# Autodesk Inventor assembly: Shoulder
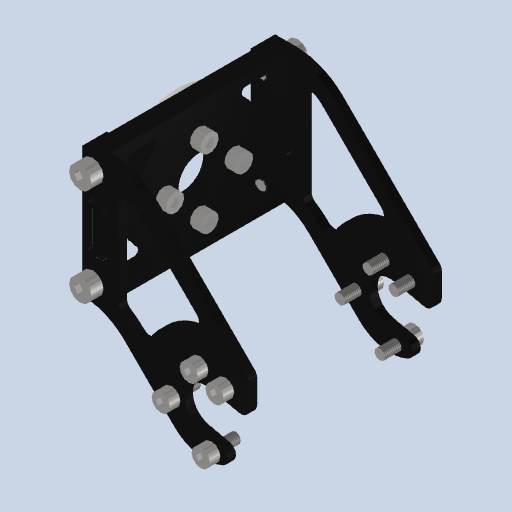
[picture p0: Inventor's stored thumbnail of the model, 512x512]
Saved by Autodesk Inventor 2022 (Build 260153000, 153)
## iProperties
Created: 2022-01-10
Part Number: Shoulder
Document SubType Name: Assembly
Designer: Masato Kubotera
Author: Masato Kubotera
## Documents named in this file (7)
- C:\Users\MasatoKubotera\Desktop\SUSTAINA-OP\UpperBody\Arm\Shoulder.iam
- C:\Users\MasatoKubotera\Desktop\SUSTAINA-OP\ReadyMade\Washer\TT-2532-10.ipt
- C:\Users\MasatoKubotera\Desktop\SUSTAINA-OP\UpperBody\Arm\Shoulder_horn_frame.ipt
- C:\Users\MasatoKubotera\Desktop\SUSTAINA-OP\UpperBody\Arm\Shoulder_side_frame.ipt
- C:\Users\MasatoKubotera\Desktop\SUSTAINA-OP\ReadyMade\Screw\UC-2606.ipt
- C:\Users\MasatoKubotera\Desktop\SUSTAINA-OP\ReadyMade\Screw\UC-2608.ipt
- C:\Users\MasatoKubotera\Desktop\SUSTAINA-OP\ReadyMade\Screw\UC-0306.ipt
## Components (20 placed, 6 different names)
1. Shoulder_horn_frame:1 — メイト:1, メイト:2, メイト:3, 挿入:1, 挿入:2, 挿入:3, 挿入:4, 挿入:5, 挿入:14, 挿入:15, 挿入:16, 挿入:17
2. Shoulder_side_frame:1 — 挿入:2, 挿入:3, 挿入:6, 挿入:7, 挿入:8, 挿入:9, 挿入:18, 挿入:19
3. Shoulder_side_frame:2 — 挿入:4, 挿入:5, 挿入:10, 挿入:11, 挿入:12, 挿入:13, 挿入:20, 挿入:21
4. TT-2532-10:1 — 挿入:1
5. UC-2606:1 — 挿入:6
6. UC-2606:2 — 挿入:7
7. UC-2606:3 — 挿入:8
8. UC-2606:4 — 挿入:9
9. UC-2606:5 — 挿入:10
10. UC-2606:6 — 挿入:11
11. UC-2606:7 — 挿入:12
12. UC-2606:8 — 挿入:13
13. UC-2608:1 — 挿入:14
14. UC-2608:2 — 挿入:15
15. UC-2608:3 — 挿入:16
16. UC-2608:4 — 挿入:17
17. UC-0306:1 — 挿入:18
18. UC-0306:2 — 挿入:19
19. UC-0306:3 — 挿入:20
20. UC-0306:4 — 挿入:21
## Relationships (24: Insert 21, Mate 3)
- メイト:1 [Mate]: Shoulder_horn_frame:1
- メイト:2 [Mate]: Shoulder_horn_frame:1
- メイト:3 [Mate]: Shoulder_horn_frame:1
- 挿入:1 [Insert]: Shoulder_horn_frame:1 ↔ TT-2532-10:1
- 挿入:2 [Insert]: Shoulder_horn_frame:1 ↔ Shoulder_side_frame:1
- 挿入:3 [Insert]: Shoulder_horn_frame:1 ↔ Shoulder_side_frame:1
- 挿入:4 [Insert]: Shoulder_horn_frame:1 ↔ Shoulder_side_frame:2
- 挿入:5 [Insert]: Shoulder_horn_frame:1 ↔ Shoulder_side_frame:2
- 挿入:6 [Insert]: Shoulder_side_frame:1 ↔ UC-2606:1
- 挿入:7 [Insert]: Shoulder_side_frame:1 ↔ UC-2606:2
- 挿入:8 [Insert]: Shoulder_side_frame:1 ↔ UC-2606:3
- 挿入:9 [Insert]: Shoulder_side_frame:1 ↔ UC-2606:4
- 挿入:10 [Insert]: Shoulder_side_frame:2 ↔ UC-2606:5
- 挿入:11 [Insert]: Shoulder_side_frame:2 ↔ UC-2606:6
- 挿入:12 [Insert]: Shoulder_side_frame:2 ↔ UC-2606:7
- 挿入:13 [Insert]: Shoulder_side_frame:2 ↔ UC-2606:8
- 挿入:14 [Insert]: Shoulder_horn_frame:1 ↔ UC-2608:1
- 挿入:15 [Insert]: Shoulder_horn_frame:1 ↔ UC-2608:2
- 挿入:16 [Insert]: Shoulder_horn_frame:1 ↔ UC-2608:3
- 挿入:17 [Insert]: Shoulder_horn_frame:1 ↔ UC-2608:4
- 挿入:18 [Insert]: Shoulder_side_frame:1 ↔ UC-0306:1
- 挿入:19 [Insert]: Shoulder_side_frame:1 ↔ UC-0306:2
- 挿入:20 [Insert]: Shoulder_side_frame:2 ↔ UC-0306:3
- 挿入:21 [Insert]: Shoulder_side_frame:2 ↔ UC-0306:4
